# Autodesk Inventor assembly: Giant-Snes-Gamepad
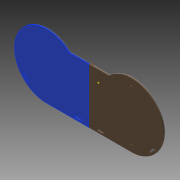
[picture p0: Inventor's stored thumbnail of the model, 180x180]
Saved by Autodesk Inventor 2014 SP1 (Build 180222100, 222)
## iProperties
Created: 2014-01-12
Part Number: Giant-Snes-Gamepad
Document SubType Name: Assembly
Designer: tuleu
Author: tuleu
## Documents named in this file (5)
- C:\Users\tuleu\Documents\giant-snes-gamepad\cad\Giant_Snes_Gamepad.iam
- C:\Users\tuleu\Documents\giant-snes-gamepad\cad\Base.ipt
- C:\Users\tuleu\Documents\giant-snes-gamepad\cad\Link.ipt
- C:\Users\tuleu\Documents\giant-snes-gamepad\cad\Gamepad_Left.iam
- C:\Users\tuleu\Documents\giant-snes-gamepad\cad\Gamepad_Right.iam
## Components (6 placed, 4 different names)
1. Base:2 — Mate:4, Flush:2, Mate:10, Mate:11, Mate:12, Mate:13, Mate:38
2. Link:1 — Mate:4, Flush:2, Mate:12
3. Link:2 — Mate:10, Mate:14
4. Link:3 — Mate:11
5. Gamepad_Left:1 [sub-assembly]
6. Gamepad_Right:1 [sub-assembly]
## Relationships (39: Mate 33, Flush 4, Angle 2)
- [Mate]: Base:2 ↔ Gamepad_Left:1
- [Mate]: Base:2 ↔ Gamepad_Left:1
- [Flush]: Base:2 ↔ Gamepad_Left:1
- [Mate]: Base:2 ↔ Gamepad_Left:1
- Mate:4: Base:2 ↔ Link:1
- [Mate]: Link:2 ↔ Gamepad_Left:1
- [Mate]: Link:3 ↔ Gamepad_Left:1
- Flush:2: Base:2 ↔ Link:1
- [Flush]: Link:3 ↔ Gamepad_Left:1
- Mate:10: Base:2 ↔ Link:2
- Mate:11: Base:2 ↔ Link:3
- Mate:12: Base:2 ↔ Link:1
- Mate:13: Base:2
- Mate:14: Link:2
- [Mate] (-205 mm): Gamepad_Left:1
- [Mate]: Base:2 ↔ Gamepad_Right:1
- [Mate]: Base:2 ↔ Gamepad_Right:1
- [Mate] (-400 mm): Base:2 ↔ Gamepad_Right:1
- [Mate]: Base:2 ↔ Gamepad_Right:1
- [Mate]: Gamepad_Left:1
- [Angle] (0 deg): Gamepad_Left:1
- [Mate]: Gamepad_Left:1
- Mate:38: Base:2
- [Angle] (0 deg): Gamepad_Left:1
- [Flush]: Gamepad_Right:1
- [Mate]: Base:2 ↔ Gamepad_Right:1
- [Mate]: Base:2 ↔ Gamepad_Right:1
- [Mate]: Base:2 ↔ Gamepad_Right:1
- [Mate]: Base:2 ↔ Gamepad_Right:1
- [Mate]: Base:2 ↔ Gamepad_Right:1
- [Mate]: Base:2 ↔ Gamepad_Right:1
- [Mate]: Base:2 ↔ Gamepad_Right:1
- [Mate] (-280 mm): Base:2 ↔ Gamepad_Right:1
- [Mate] (-280 mm): Base:2 ↔ Gamepad_Right:1
- [Mate] (-280 mm): Base:2 ↔ Gamepad_Right:1
- [Mate] (-280 mm): Base:2 ↔ Gamepad_Right:1
- [Mate]: Base:2 ↔ Gamepad_Right:1
- [Mate]: Base:2 ↔ Gamepad_Right:1
- [Mate]: Base:2 ↔ Gamepad_Right:1
